# Autodesk Inventor assembly: !structure_half_mirrored
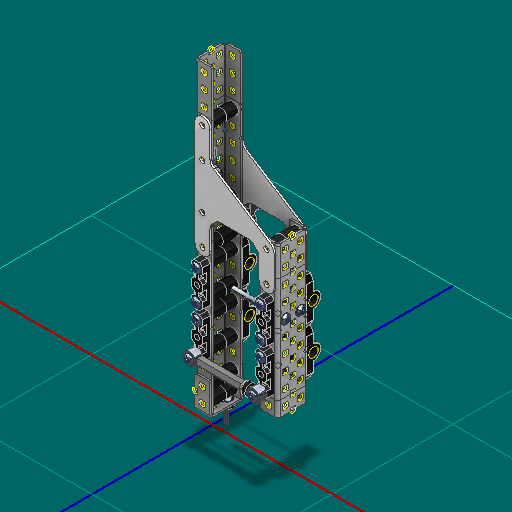
[picture p0: Inventor's stored thumbnail of the model, 512x512]
Saved by Autodesk Inventor 2025 (Build 290162000, 162)
## iProperties
Created: 2024-08-20
Part Number: !structure_half_mirrored
Document SubType Name: Assembly
Designer: averey
Author: averey
## Documents named in this file (21)
- C:\Users\avere\vex_robotics_high_stakes\hardware\cad\ATLAS\tower\structure\structure_half_mirrored\!structure_half_mirrored.iam
- C:\Users\avere\vex_robotics_high_stakes\hardware\cad\ATLAS\tower\structure\structure_half_mirrored\structure_channel_mirrored.iam
- C:\Users\avere\vex_robotics_high_stakes\hardware\cad\ATLAS\tower\structure\structure_half_mirrored\intake_gearbox_outer_mirrored.iam
- C:\Users\avere\vex_robotics_high_stakes\hardware\cad\ATLAS\tower\structure\structure_half_mirrored\Bearing Flat Low Profile 2-Hole_mirrored.ipt
- C:\Users\avere\vex_robotics_high_stakes\hardware\cad\VEX-CAD-Inventor\Structure\Hardware\Screw Steel - Star\SScrew Star Smooth 1.750.ipt
- C:\Users\avere\vex_robotics_high_stakes\hardware\cad\VEX-CAD-Inventor\Structure\Hardware\Screw Steel - Star.ipt
- C:\Users\avere\vex_robotics_high_stakes\hardware\cad\VEX-CAD-Inventor\Structure\Hardware\Screw Shoulder Robosource\SScrew Shoulder Smooth .500 x .04.ipt
- C:\Users\avere\vex_robotics_high_stakes\hardware\cad\VEX-CAD-Inventor\Structure\Hardware\Screw Shoulder Robosource.ipt
- C:\Users\avere\vex_robotics_high_stakes\hardware\cad\ATLAS\tower\structure\structure_half_mirrored\Nut Thin Nylock_mirrored.ipt
- C:\Users\avere\vex_robotics_high_stakes\hardware\cad\ATLAS\tower\structure\structure_half_mirrored\gusset_mirrored.ipt
- C:\Users\avere\vex_robotics_high_stakes\hardware\cad\ATLAS\tower\structure\structure_half_mirrored\LS Pillow Bearing Block_mirrored.ipt
- C:\Users\avere\vex_robotics_high_stakes\hardware\cad\VEX-CAD-Inventor\Motion\Spacers\Spacer Nylon .375 OD\NSpacer .375 OD x .250.ipt
- C:\Users\avere\vex_robotics_high_stakes\hardware\cad\VEX-CAD-Inventor\Motion\Spacers\Spacer Nylon .375 OD.ipt
- C:\Users\avere\vex_robotics_high_stakes\hardware\cad\VEX-CAD-Inventor\Motion\Spacers\Washer Steel\SWasher .375 OD x .015625.ipt
- C:\Users\avere\vex_robotics_high_stakes\hardware\cad\VEX-CAD-Inventor\Motion\Spacers\Washer Steel.ipt
- C:\Users\avere\vex_robotics_high_stakes\hardware\cad\VEX-CAD-Inventor\Motion\Spacers\Washer Steel\SWasher .375 OD x .031250.ipt
- C:\Users\avere\vex_robotics_high_stakes\hardware\cad\VEX-CAD-Inventor\Motion\Spacers\Washer Steel\SWasher .375 OD x .062500.ipt
- C:\Users\avere\vex_robotics_high_stakes\hardware\cad\ATLAS\tower\structure\structure_half_mirrored\Shaft Collar No Screw_mirrored.ipt
- C:\Users\avere\vex_robotics_high_stakes\hardware\cad\VEX-CAD-Inventor\Motion\Spacers\Spacer Nylon .375 OD\NSpacer .375 OD x .125.ipt
- C:\Users\avere\vex_robotics_high_stakes\hardware\cad\VEX-CAD-Inventor\Structure\Standoff\Standoff 1.50.ipt
- C:\Users\avere\vex_robotics_high_stakes\hardware\cad\VEX-CAD-Inventor\Structure\Standoff.ipt
## Components (22 placed, 15 different names)
1. structure_channel_mirrored:1 [sub-assembly] — Mate:8, Mate:1, Insert:6, Mate:4, Insert:18
2. intake_gearbox_outer_mirrored:1 [sub-assembly] — Angle:2, Mate:1, Insert:1, Mate:2, Insert:2, Insert:4, Insert:16, Mate:6, Insert:17
3. Bearing Flat Low Profile 2-Hole_mirrored:1 — Insert:1, Mate:2, Insert:3
4. SScrew Star Smooth 1.750:1 — Insert:2
5. SScrew Shoulder Smooth .500 x .04:1 — Insert:4
6. Nut Thin Nylock_mirrored:1 — Insert:3
7. gusset_mirrored:1 — Insert:5, Mate:3
8. gusset_mirrored:2 — Angle:1, Insert:16, Insert:6, Insert:5, Mate:6, Mate:4, Mate:3, Insert:22, Mate:9
9. LS Pillow Bearing Block_mirrored:1 — Insert:14, Insert:13
10. NSpacer .375 OD x .250:1 — Insert:7, Mate:9
11. SWasher .375 OD x .015625:1 — Insert:14, Insert:9
12. SWasher .375 OD x .031250:2 — Insert:9, Insert:8
13. SWasher .375 OD x .062500:3 — Insert:8, Insert:7
14. NSpacer .375 OD x .250:2 — Insert:10, Insert:22
15. SWasher .375 OD x .015625:4 — Insert:13, Insert:12
16. SWasher .375 OD x .031250:5 — Insert:12, Insert:11
17. SWasher .375 OD x .062500:6 — Insert:11, Insert:10
18. Shaft Collar No Screw_mirrored:1 — Insert:17, Mate:7, Insert:21
19. Shaft Collar No Screw_mirrored:2 — Insert:18, Mate:7
20. NSpacer .375 OD x .125:3 — Insert:21, Insert:19
21. SWasher .375 OD x .062500:7 — Insert:19, Insert:20
22. Standoff 1.50:1 — Insert:20
## Relationships (31: Insert 21, Mate 8, Angle 2)
- Mate:8: structure_channel_mirrored:1
- Angle:2 (0 deg): intake_gearbox_outer_mirrored:1
- Mate:1: structure_channel_mirrored:1 ↔ intake_gearbox_outer_mirrored:1
- Insert:1: intake_gearbox_outer_mirrored:1 ↔ Bearing Flat Low Profile 2-Hole_mirrored:1
- Mate:2: intake_gearbox_outer_mirrored:1 ↔ Bearing Flat Low Profile 2-Hole_mirrored:1
- Insert:2: intake_gearbox_outer_mirrored:1 ↔ SScrew Star Smooth 1.750:1
- Insert:4: intake_gearbox_outer_mirrored:1 ↔ SScrew Shoulder Smooth .500 x .04:1
- Insert:3 (1.27 mm): Bearing Flat Low Profile 2-Hole_mirrored:1 ↔ Nut Thin Nylock_mirrored:1
- Angle:1 (0 deg): gusset_mirrored:2
- Insert:16: intake_gearbox_outer_mirrored:1 ↔ gusset_mirrored:2
- Insert:6: structure_channel_mirrored:1 ↔ gusset_mirrored:2
- Insert:5 (25.4 mm): gusset_mirrored:1 ↔ gusset_mirrored:2
- Mate:6: intake_gearbox_outer_mirrored:1 ↔ gusset_mirrored:2
- Mate:4: structure_channel_mirrored:1 ↔ gusset_mirrored:2
- Mate:3: gusset_mirrored:1 ↔ gusset_mirrored:2
- Insert:14: LS Pillow Bearing Block_mirrored:1 ↔ SWasher .375 OD x .015625:1
- Insert:9: SWasher .375 OD x .015625:1 ↔ SWasher .375 OD x .031250:2
- Insert:8: SWasher .375 OD x .031250:2 ↔ SWasher .375 OD x .062500:3
- Insert:7: NSpacer .375 OD x .250:1 ↔ SWasher .375 OD x .062500:3
- Insert:13: LS Pillow Bearing Block_mirrored:1 ↔ SWasher .375 OD x .015625:4
- Insert:12: SWasher .375 OD x .015625:4 ↔ SWasher .375 OD x .031250:5
- Insert:11: SWasher .375 OD x .031250:5 ↔ SWasher .375 OD x .062500:6
- Insert:10: NSpacer .375 OD x .250:2 ↔ SWasher .375 OD x .062500:6
- Insert:17: intake_gearbox_outer_mirrored:1 ↔ Shaft Collar No Screw_mirrored:1
- Insert:18: structure_channel_mirrored:1 ↔ Shaft Collar No Screw_mirrored:2
- Mate:7: Shaft Collar No Screw_mirrored:1 ↔ Shaft Collar No Screw_mirrored:2
- Insert:21: Shaft Collar No Screw_mirrored:1 ↔ NSpacer .375 OD x .125:3
- Insert:19: NSpacer .375 OD x .125:3 ↔ SWasher .375 OD x .062500:7
- Insert:20: SWasher .375 OD x .062500:7 ↔ Standoff 1.50:1
- Insert:22: gusset_mirrored:2 ↔ NSpacer .375 OD x .250:2
- Mate:9: gusset_mirrored:2 ↔ NSpacer .375 OD x .250:1
